# Autodesk Inventor assembly: Pen_Plotter
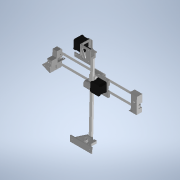
[picture p0: Inventor's stored thumbnail of the model, 180x180]
Saved by Autodesk Inventor 2021 (Build 250183000, 183)
## iProperties
Created: 2021-03-29
Part Number: Pen_Plotter
Document SubType Name: Assembly
Designer: Ariel Wolle
Author: Ariel Wolle
## Documents named in this file (11)
- D:\Documents\dev\Project-4\Pen_Plotter.iam
- D:\Documents\dev\Project-4\350mm_linear_rod.ipt
- D:\Documents\dev\Project-4\Imported Components\RaftMount\RaftMount.ipt
- D:\Documents\dev\Project-4\Imported Components\BaseEnd-Idle\BaseEnd-Idle.ipt
- D:\Documents\dev\Project-4\Imported Components\BaseEnd-Powered\BaseEnd-Powered.ipt
- D:\Documents\dev\Project-4\Linear_Rail_Basic.ipt
- D:\Documents\dev\Project-4\Linear_Rail_Carrier_Basic.ipt
- D:\Documents\dev\Project-4\Imported Components\Y-Pen-End\Y-Pen-End.ipt
- D:\Documents\dev\Project-4\Imported Components\Y-Servo-Housing\Y-Servo-Housing.ipt
- D:\Documents\dev\Project-4\Imported Components\PenSlider\PenSlider.ipt
- D:\Documents\dev\Project-4\Imported Components\Motor_NEMA17\Motor_NEMA17.ipt
## Components (12 placed, 10 different names)
1. 350mm_linear_rod:1 — Mate:1, Flush:1, Mate:16, Mate:21, Mate:22
2. 350mm_linear_rod:2 — Mate:2, Flush:1, Mate:15, Mate:17, Mate:20
3. RaftMount:1 — Mate:1, Mate:2, Mate:11, Mate:12, Mate:13, Mate:14, Mate:25, Mate:26, Angle:2
4. BaseEnd-Idle:1 — Mate:3, Mate:4, Mate:5
5. BaseEnd-Powered:1 — Mate:6, Mate:7, Mate:8, Mate:23, Mate:24, Angle:1
6. Linear_Rail_Basic:1 — Mate:3, Mate:4, Mate:5, Mate:6, Mate:7, Mate:8, Mate:9, Mate:10
7. Linear_Rail_Carrier_Basic:1 — Mate:9, Mate:10, Mate:11, Mate:12, Mate:13, Mate:14
8. Y-Pen-End:1 — Mate:18, Mate:19, Mate:20, Mate:21, Mate:22
9. Y-Servo-Housing:1 — Mate:15, Mate:16, Mate:17
10. PenSlider:1 — Mate:18, Mate:19
11. Motor_NEMA17:1 — Mate:25, Mate:26, Angle:2
12. Motor_NEMA17:3 — Mate:23, Mate:24, Angle:1
## Relationships (29: Mate 26, Angle 2, Flush 1)
- Mate:1: 350mm_linear_rod:1 ↔ RaftMount:1
- Mate:2: 350mm_linear_rod:2 ↔ RaftMount:1
- Mate:3: BaseEnd-Idle:1 ↔ Linear_Rail_Basic:1
- Mate:4: BaseEnd-Idle:1 ↔ Linear_Rail_Basic:1
- Mate:5: BaseEnd-Idle:1 ↔ Linear_Rail_Basic:1
- Mate:6: BaseEnd-Powered:1 ↔ Linear_Rail_Basic:1
- Mate:7: BaseEnd-Powered:1 ↔ Linear_Rail_Basic:1
- Mate:8: BaseEnd-Powered:1 ↔ Linear_Rail_Basic:1
- Mate:9: Linear_Rail_Basic:1 ↔ Linear_Rail_Carrier_Basic:1
- Mate:10: Linear_Rail_Basic:1 ↔ Linear_Rail_Carrier_Basic:1
- Mate:11: RaftMount:1 ↔ Linear_Rail_Carrier_Basic:1
- Mate:12: RaftMount:1 ↔ Linear_Rail_Carrier_Basic:1
- Mate:13: RaftMount:1 ↔ Linear_Rail_Carrier_Basic:1
- Mate:14: RaftMount:1 ↔ Linear_Rail_Carrier_Basic:1
- Flush:1: 350mm_linear_rod:1 ↔ 350mm_linear_rod:2
- Mate:15: 350mm_linear_rod:2 ↔ Y-Servo-Housing:1
- Mate:16: 350mm_linear_rod:1 ↔ Y-Servo-Housing:1
- Mate:17: 350mm_linear_rod:2 ↔ Y-Servo-Housing:1
- Mate:18: Y-Pen-End:1 ↔ PenSlider:1
- Mate:19 (-1 mm): Y-Pen-End:1 ↔ PenSlider:1
- Mate:20: 350mm_linear_rod:2 ↔ Y-Pen-End:1
- Mate:21: 350mm_linear_rod:1 ↔ Y-Pen-End:1
- Mate:22: 350mm_linear_rod:1 ↔ Y-Pen-End:1
- Mate:23: BaseEnd-Powered:1 ↔ Motor_NEMA17:3
- Mate:24: BaseEnd-Powered:1 ↔ Motor_NEMA17:3
- Angle:1 (0 deg): BaseEnd-Powered:1 ↔ Motor_NEMA17:3
- Mate:25: RaftMount:1 ↔ Motor_NEMA17:1
- Mate:26: RaftMount:1 ↔ Motor_NEMA17:1
- Angle:2 (0 deg): RaftMount:1 ↔ Motor_NEMA17:1
